# Autodesk Inventor assembly: CrossBarAssembly
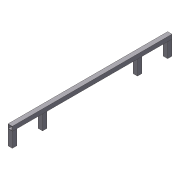
[picture p0: Inventor's stored thumbnail of the model, 180x180]
Saved by Autodesk Inventor 2012 (Build 160160000, 160)
## iProperties
Created: 2012-01-20
Part Number: CrossBarAssembly
Document SubType Name: Assembly
Designer: JesseK
Author: JesseK
## Documents named in this file (3)
- Z:\UserData\Documents\Inventor\team1885frc\Robot2012\Drawings\CrossBarAssembly.iam
- Z:\UserData\Documents\Inventor\team1885frc\Robot2012\DriveTrain\Frame_FrontVerticalSupport_forFrontCrossbar.ipt
- Z:\UserData\Documents\Inventor\team1885frc\Robot2012\DriveTrain\Frame_LongCrossMember.ipt
## Components (5 placed, 2 different names)
1. Frame_FrontVerticalSupport_forFrontCrossbar:1 — Mate:8, Flush:3, Mate:12, Mate:13
2. Frame_FrontVerticalSupport_forFrontCrossbar:2 — Mate:8, Flush:2, Flush:3, Mate:11
3. Frame_FrontVerticalSupport_forFrontCrossbar:3 — Mate:7, Flush:1, Flush:2, Mate:14
4. Frame_FrontVerticalSupport_forFrontCrossbar:4 — Mate:7, Mate:9, Flush:1, Flush:4, Mate:10
5. Frame_LongCrossMember:1 — Mate:9, Flush:4, Mate:10, Mate:11, Mate:12, Mate:13, Mate:14
## Relationships (12: Mate 8, Flush 4)
- Mate:7 (152.4 mm): Frame_FrontVerticalSupport_forFrontCrossbar:3 ↔ Frame_FrontVerticalSupport_forFrontCrossbar:4
- Mate:8 (152.4 mm): Frame_FrontVerticalSupport_forFrontCrossbar:1 ↔ Frame_FrontVerticalSupport_forFrontCrossbar:2
- Mate:9: Frame_FrontVerticalSupport_forFrontCrossbar:4 ↔ Frame_LongCrossMember:1
- Flush:1: Frame_FrontVerticalSupport_forFrontCrossbar:3 ↔ Frame_FrontVerticalSupport_forFrontCrossbar:4
- Flush:2: Frame_FrontVerticalSupport_forFrontCrossbar:2 ↔ Frame_FrontVerticalSupport_forFrontCrossbar:3
- Flush:3: Frame_FrontVerticalSupport_forFrontCrossbar:1 ↔ Frame_FrontVerticalSupport_forFrontCrossbar:2
- Flush:4: Frame_FrontVerticalSupport_forFrontCrossbar:4 ↔ Frame_LongCrossMember:1
- Mate:10: Frame_FrontVerticalSupport_forFrontCrossbar:4 ↔ Frame_LongCrossMember:1
- Mate:11: Frame_FrontVerticalSupport_forFrontCrossbar:2 ↔ Frame_LongCrossMember:1
- Mate:12: Frame_FrontVerticalSupport_forFrontCrossbar:1 ↔ Frame_LongCrossMember:1
- Mate:13: Frame_FrontVerticalSupport_forFrontCrossbar:1 ↔ Frame_LongCrossMember:1
- Mate:14: Frame_FrontVerticalSupport_forFrontCrossbar:3 ↔ Frame_LongCrossMember:1
